# Autodesk Inventor assembly: leftArm
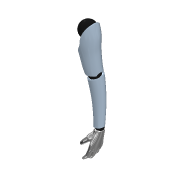
[picture p0: Inventor's stored thumbnail of the model, 180x180]
Saved by Autodesk Inventor 2021 (Build 250183000, 183)
## iProperties
Created: 2021-03-28
Part Number: leftArm
Document SubType Name: Assembly
Designer: Derm
Author: Derm
## Documents named in this file (2)
- C:\Users\Derm\roboticArm\humanPoseEstimation\human\leftArm.iam
- C:\Users\Derm\roboticArm\multibodySim\human\Corpo Humano - ADEBOTT Projetos\01.02.03.00 - Braço esquerdo.iam
## Components (1 placed, 1 different names)
1. 01.02.03.00 - Braço esquerdo:1 [sub-assembly] — Flush:1, Flush:2, Flush:3
## Relationships (3: Flush 3)
- Flush:1 (196.85 mm): 01.02.03.00 - Braço esquerdo:1
- Flush:2 (-45.72 mm): 01.02.03.00 - Braço esquerdo:1
- Flush:3 (1384.3 mm): 01.02.03.00 - Braço esquerdo:1
